# Autodesk Inventor assembly: SpiritBot V1.0
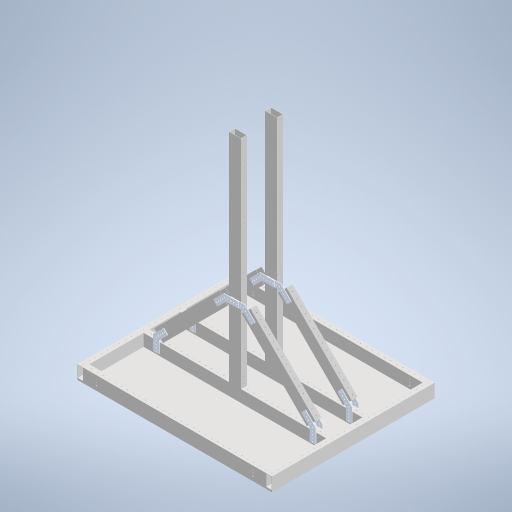
[picture p0: Inventor's stored thumbnail of the model, 512x512]
Saved by Autodesk Inventor 2024 (Build 280153000, 153)
## iProperties
Created: 2023-07-06
Part Number: SpiritBot V1.0
Document SubType Name: Assembly
Designer: Gabriel Marquez
Author: Gabriel Marquez
## Documents named in this file (8)
- C:\Users\Gabriel Marquez\OneDrive\Documents\GitHub\T3-CAD\Current Season CAD\SpiritBot V1.0.iam
- C:\Users\Gabriel Marquez\OneDrive\Documents\GitHub\T3-CAD\Current Season CAD\Body\Base.ipt
- C:\Users\Gabriel Marquez\OneDrive\Documents\GitHub\T3-CAD\Current Season CAD\Body\Long bar 3- VersaFrame.ipt
- C:\Users\Gabriel Marquez\OneDrive\Documents\GitHub\T3-CAD\Current Season CAD\Body\Long bar 4- VersaFrame.ipt
- C:\Users\Gabriel Marquez\OneDrive\Documents\GitHub\T3-CAD\Current Season CAD\Body\Long bar 8.5 - VersaFrame.ipt
- C:\Users\Gabriel Marquez\OneDrive\Documents\GitHub\T3-CAD\Current Season CAD\Body\Long bar 32.3 - VersaFrame.ipt
- C:\Users\Gabriel Marquez\OneDrive\Documents\GitHub\T3-CAD\Stock\Versa System\Gussets\135 Degree Gusset.ipt
- C:\Users\Gabriel Marquez\OneDrive\Documents\GitHub\T3-CAD\Current Season CAD\Body\cut gusset.ipt
## Components (27 placed, 7 different names)
1. Base:1 — Mate:7, Mate:8
2. Long bar 32.3 - VersaFrame:1 — Mate:1, Mate:2, Mate:6, Mate:7, Mate:14
3. Long bar 32.3 - VersaFrame:2 — Mate:5, Mate:26
4. Long bar 32.3 - VersaFrame:3 — Mate:10, Mate:11, Mate:14, Mate:15, Mate:16, Rotational:7, Rotational:8, Rotational:17, Rotational:18
5. Long bar 8.5 - VersaFrame:1 — Mate:1, Mate:2, Mate:5, Mate:11, Mate:24
6. Long bar 8.5 - VersaFrame:2 — Mate:6, Mate:8, Mate:10, Mate:20, Mate:23
7. Long bar 3- VersaFrame:2 — Mate:15, Mate:16, Mate:20, Rotational:1, Rotational:2, Mate:25
8. Long bar 4- VersaFrame:1 — Rotational:3, Rotational:4, Rotational:5, Rotational:6
9. 135 Degree Gusset:1 — Rotational:1, Rotational:2, Rotational:9, Rotational:10
10. 135 Degree Gusset:3 — Rotational:5, Rotational:6, Rotational:7, Rotational:8
11. 135 Degree Gusset:4 — Rotational:3, Rotational:4
12. 135 Degree Gusset:5 — Rotational:9, Rotational:10, Rotational:11, Rotational:12
13. cut gusset:1 — Rotational:11, Rotational:12
14. Long bar 4- VersaFrame:2
15. 135 Degree Gusset:6
16. 135 Degree Gusset:7 — Rotational:17, Rotational:18
17. Long bar 4- VersaFrame:3
18. Long bar 32.3 - VersaFrame:4 — Mate:23, Mate:24, Mate:26
19. Long bar 3- VersaFrame:3 — Mate:25
20. 135 Degree Gusset:8
21. 135 Degree Gusset:9
22. 135 Degree Gusset:10
23. 135 Degree Gusset:11
24. cut gusset:2
25. Long bar 4- VersaFrame:4
26. 135 Degree Gusset:12
27. 135 Degree Gusset:13
## Relationships (56: RevoluteJoint 36, Mate 20)
- Mate:1: Long bar 32.3 - VersaFrame:1 ↔ Long bar 8.5 - VersaFrame:1
- Mate:2: Long bar 32.3 - VersaFrame:1 ↔ Long bar 8.5 - VersaFrame:1
- [Mate]: Long bar 32.3 - VersaFrame:2 ↔ Long bar 8.5 - VersaFrame:2
- [Mate]: Long bar 32.3 - VersaFrame:2 ↔ Long bar 8.5 - VersaFrame:2
- Mate:5: Long bar 32.3 - VersaFrame:2 ↔ Long bar 8.5 - VersaFrame:1
- Mate:6: Long bar 32.3 - VersaFrame:1 ↔ Long bar 8.5 - VersaFrame:2
- Mate:7: Base:1 ↔ Long bar 32.3 - VersaFrame:1
- Mate:8: Base:1 ↔ Long bar 8.5 - VersaFrame:2
- Mate:10: Long bar 32.3 - VersaFrame:3 ↔ Long bar 8.5 - VersaFrame:2
- Mate:11: Long bar 32.3 - VersaFrame:3 ↔ Long bar 8.5 - VersaFrame:1
- Mate:14 (228.6 mm): Long bar 32.3 - VersaFrame:1 ↔ Long bar 32.3 - VersaFrame:3
- Mate:15: Long bar 32.3 - VersaFrame:3 ↔ Long bar 3- VersaFrame:2
- Mate:16: Long bar 32.3 - VersaFrame:3 ↔ Long bar 3- VersaFrame:2
- Mate:20 (359.41 mm): Long bar 8.5 - VersaFrame:2 ↔ Long bar 3- VersaFrame:2
- Rotational:1 [RevoluteJoint]: Long bar 3- VersaFrame:2 ↔ 135 Degree Gusset:1
- Rotational:2 [RevoluteJoint]: Long bar 3- VersaFrame:2 ↔ 135 Degree Gusset:1
- Rotational:3 [RevoluteJoint]: Long bar 4- VersaFrame:1 ↔ 135 Degree Gusset:4
- Rotational:4 [RevoluteJoint]: Long bar 4- VersaFrame:1 ↔ 135 Degree Gusset:4
- Rotational:5 [RevoluteJoint]: Long bar 4- VersaFrame:1 ↔ 135 Degree Gusset:3
- Rotational:6 [RevoluteJoint]: Long bar 4- VersaFrame:1 ↔ 135 Degree Gusset:3
- Rotational:7 [RevoluteJoint]: Long bar 32.3 - VersaFrame:3 ↔ 135 Degree Gusset:3
- Rotational:8 [RevoluteJoint]: Long bar 32.3 - VersaFrame:3 ↔ 135 Degree Gusset:3
- Rotational:9 [RevoluteJoint]: 135 Degree Gusset:1 ↔ 135 Degree Gusset:5
- Rotational:10 [RevoluteJoint]: 135 Degree Gusset:1 ↔ 135 Degree Gusset:5
- Rotational:11 [RevoluteJoint]: 135 Degree Gusset:5 ↔ cut gusset:1
- Rotational:12 [RevoluteJoint]: 135 Degree Gusset:5 ↔ cut gusset:1
- [RevoluteJoint]: Long bar 4- VersaFrame:2 ↔ 135 Degree Gusset:7
- [RevoluteJoint]: Long bar 4- VersaFrame:2 ↔ 135 Degree Gusset:7
- [RevoluteJoint]: Long bar 4- VersaFrame:2 ↔ 135 Degree Gusset:6
- [RevoluteJoint]: Long bar 4- VersaFrame:2 ↔ 135 Degree Gusset:6
- Rotational:17 [RevoluteJoint]: Long bar 32.3 - VersaFrame:3 ↔ 135 Degree Gusset:7
- Rotational:18 [RevoluteJoint]: Long bar 32.3 - VersaFrame:3 ↔ 135 Degree Gusset:7
- [Mate]: Long bar 32.3 - VersaFrame:4 ↔ Long bar 3- VersaFrame:3
- [Mate]: Long bar 32.3 - VersaFrame:4 ↔ Long bar 3- VersaFrame:3
- [RevoluteJoint]: Long bar 3- VersaFrame:3 ↔ 135 Degree Gusset:8
- [RevoluteJoint]: Long bar 3- VersaFrame:3 ↔ 135 Degree Gusset:8
- [RevoluteJoint]: Long bar 4- VersaFrame:3 ↔ 135 Degree Gusset:10
- [RevoluteJoint]: Long bar 4- VersaFrame:3 ↔ 135 Degree Gusset:10
- [RevoluteJoint]: Long bar 4- VersaFrame:3 ↔ 135 Degree Gusset:9
- [RevoluteJoint]: Long bar 4- VersaFrame:3 ↔ 135 Degree Gusset:9
- [RevoluteJoint]: Long bar 32.3 - VersaFrame:4 ↔ 135 Degree Gusset:9
- [RevoluteJoint]: Long bar 32.3 - VersaFrame:4 ↔ 135 Degree Gusset:9
- [RevoluteJoint]: 135 Degree Gusset:8 ↔ 135 Degree Gusset:11
- [RevoluteJoint]: 135 Degree Gusset:8 ↔ 135 Degree Gusset:11
- [RevoluteJoint]: 135 Degree Gusset:11 ↔ cut gusset:2
- [RevoluteJoint]: 135 Degree Gusset:11 ↔ cut gusset:2
- [RevoluteJoint]: Long bar 4- VersaFrame:4 ↔ 135 Degree Gusset:13
- [RevoluteJoint]: Long bar 4- VersaFrame:4 ↔ 135 Degree Gusset:13
- [RevoluteJoint]: Long bar 4- VersaFrame:4 ↔ 135 Degree Gusset:12
- [RevoluteJoint]: Long bar 4- VersaFrame:4 ↔ 135 Degree Gusset:12
- [RevoluteJoint]: Long bar 32.3 - VersaFrame:4 ↔ 135 Degree Gusset:13
- [RevoluteJoint]: Long bar 32.3 - VersaFrame:4 ↔ 135 Degree Gusset:13
- Mate:23: Long bar 8.5 - VersaFrame:2 ↔ Long bar 32.3 - VersaFrame:4
- Mate:24: Long bar 8.5 - VersaFrame:1 ↔ Long bar 32.3 - VersaFrame:4
- Mate:25: Long bar 3- VersaFrame:2 ↔ Long bar 3- VersaFrame:3
- Mate:26 (228.6 mm): Long bar 32.3 - VersaFrame:2 ↔ Long bar 32.3 - VersaFrame:4
## Named parameters: d2_d0 = 0 mm, d3_d1 = 0 mm, d50_d28 = 0 mm, d51_d29 = 0 deg, d52_d32 = 0 mm, d53_d33 = 90 deg, d54_d34 = 0 mm, d55_d35 = 90 deg, d56_d36 = 0 mm, d57_d37 = 90 deg, d62_d14 = 0 mm, d63_d15 = 0 mm, d64_d20 = 0 mm, d65_d21 = -45 deg, d66_d22 = 0 mm, d67_d23 = -45 deg, d68_d28 = 0 mm, d69_d29 = 0 deg, d70_d32 = 0 mm, d71_d33 = 90 deg, d72_d34 = 0 mm, d73_d35 = 90 deg, d74_d36 = 0 mm, d75_d37 = 90 deg, d76_d38 = 0 mm, d77_d39 = -45 deg, d78_d40 = 0 mm, d79_d41 = 135 deg, d80_d42 = 0 mm, d81_d43 = 45 deg, d82_d44 = 0 mm, d83_d45 = 45 deg, d84_d46 = 0 mm, d85_d47 = 0 deg, d86_d48 = 0 mm, d87_d49 = 180 deg, d88_d50_d28 = 0 mm, d89_d51_d29 = 0 deg, d90_d52_d32 = 0 mm, d91_d53_d33 = 90 deg, d92_d54_d34 = 0 mm, d93_d55_d35 = 90 deg, d94_d56_d36 = 0 mm, d95_d57_d37 = 90 deg, d96_d58 = 0 mm, d97_d59 = 135 deg, d98_d60 = 0 mm, d99_d61 = 135 deg
